# Autodesk Inventor assembly: derived_drive_assembly_10_1_nn32
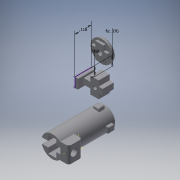
[picture p0: Inventor's stored thumbnail of the model, 180x180]
Saved by Autodesk Inventor 2016 (Build 200138000, 138)
## iProperties
Created: 2016-08-02
Part Number: derived_drive_assembly_10_1_nn32
Document SubType Name: Assembly
Designer: GentnerLab
Author: GentnerLab
## Documents named in this file (7)
- C:\Users\GentnerLab\Desktop\printable_drive\derived_drive_assembly_10_1_nn32.iam
- C:\Users\GentnerLab\Desktop\printable_drive\derived_body-10mm.ipt
- C:\Users\GentnerLab\Desktop\printable_drive\derived_shuttle_10mm.ipt
- C:\Users\GentnerLab\Desktop\printable_drive\derived_top_1mm.ipt
- C:\Users\GentnerLab\Desktop\printable_drive\probe_carrier_nn32.ipt
- C:\Users\GentnerLab\Desktop\printable_drive\derived_drive_handle.ipt
- C:\Users\GentnerLab\Documents\Inventor\Parts\new_drive\60unm-6mm\stand.ipt
## Components (8 placed, 6 different names)
1. derived_body-10mm:1 — Mate:1, Mate:7, Mate:8, Mate:9, Mate:10
2. derived_shuttle_10mm:1 — Flush:1, Mate:3, Mate:5, Mate:6
3. derived_top_1mm:1 — Mate:2
4. probe_carrier_nn32:1 — Mate:3, Mate:5, Mate:6
5. derived_drive_handle:1 — Mate:7, Mate:8, Mate:9
6. stand:1 — Mate:10
7. stand:2
8. stand:4
## Component patterns: (4 elements, first: stand:1)
## Relationships (10: Mate 9, Flush 1)
- Mate:1: derived_body-10mm:1
- Mate:2: derived_top_1mm:1
- Flush:1: derived_shuttle_10mm:1
- Mate:3: derived_shuttle_10mm:1 ↔ probe_carrier_nn32:1
- Mate:5 (0.364 mm): derived_shuttle_10mm:1 ↔ probe_carrier_nn32:1
- Mate:6: derived_shuttle_10mm:1 ↔ probe_carrier_nn32:1
- Mate:7: derived_body-10mm:1 ↔ derived_drive_handle:1
- Mate:8: derived_body-10mm:1 ↔ derived_drive_handle:1
- Mate:9 (2 mm): derived_body-10mm:1 ↔ derived_drive_handle:1
- Mate:10: derived_body-10mm:1 ↔ stand:1
